# Autodesk Inventor assembly: Assembly_FINAL
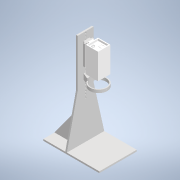
[picture p0: Inventor's stored thumbnail of the model, 180x180]
Saved by Autodesk Inventor 2021.2 (Build 252289000, 289)
## iProperties
Created: 2021-03-24
Part Number: Assembly_FINAL
Document SubType Name: Assembly
Designer: yxion
Author: yxion
## Documents named in this file (9)
- C:\Users\yxion\Documents\6_VandyUndergrad\4_ProgramManagement\EVD\CAD\Assembly_FINAL.iam
- C:\Users\yxion\Documents\6_VandyUndergrad\4_ProgramManagement\EVD\CAD\mdf_base_6x6.ipt
- C:\Users\yxion\Documents\6_VandyUndergrad\4_ProgramManagement\EVD\CAD\camera.ipt
- C:\Users\yxion\Documents\6_VandyUndergrad\4_ProgramManagement\EVD\CAD\mdf_support.ipt
- C:\Users\yxion\Documents\6_VandyUndergrad\4_ProgramManagement\EVD\CAD\5mm_bolt.ipt
- C:\Users\yxion\Documents\6_VandyUndergrad\4_ProgramManagement\EVD\CAD\ring_light_holder.ipt
- C:\Users\yxion\Documents\6_VandyUndergrad\4_ProgramManagement\EVD\CAD\mdf_vertical_r1.ipt
- C:\Users\yxion\Documents\6_VandyUndergrad\4_ProgramManagement\EVD\CAD\5mm_bolt_short.ipt
- C:\Users\yxion\Documents\6_VandyUndergrad\4_ProgramManagement\EVD\CAD\spacer_final.ipt
## Components (11 placed, 8 different names)
1. mdf_base_6x6:1 — Mate:10, Mate:13, Mate:15, Mate:16, Flush:2, Mate:17, Mate:18, Mate:19, Mate:20
2. camera:1 — Mate:30, Mate:42, Flush:3, Mate:43
3. mdf_support:1 — Mate:15, Mate:16, Mate:19
4. mdf_support:2 — Mate:10, Mate:13, Mate:20
5. 5mm_bolt:3 — Mate:26, Mate:28, Mate:30
6. 5mm_bolt:4 — Mate:25, Mate:27
7. ring_light_holder:1 — Mate:36, Mate:41
8. mdf_vertical_r1:1 — Flush:2, Mate:17, Mate:18, Mate:25, Mate:26, Mate:27, Mate:28, Mate:36, Mate:37, Mate:38, Mate:39, Mate:40
9. 5mm_bolt_short:1 — Mate:37, Mate:39, Mate:41
10. 5mm_bolt_short:2 — Mate:38, Mate:40
11. spacer_final:1 — Mate:42, Flush:3, Mate:43
## Relationships (23: Mate 21, Flush 2)
- Mate:10: mdf_base_6x6:1 ↔ mdf_support:2
- Mate:13: mdf_base_6x6:1 ↔ mdf_support:2
- Mate:15: mdf_base_6x6:1 ↔ mdf_support:1
- Mate:16: mdf_base_6x6:1 ↔ mdf_support:1
- Flush:2: mdf_base_6x6:1 ↔ mdf_vertical_r1:1
- Mate:17: mdf_base_6x6:1 ↔ mdf_vertical_r1:1
- Mate:18: mdf_base_6x6:1 ↔ mdf_vertical_r1:1
- Mate:19: mdf_base_6x6:1 ↔ mdf_support:1
- Mate:20: mdf_base_6x6:1 ↔ mdf_support:2
- Mate:25: 5mm_bolt:4 ↔ mdf_vertical_r1:1
- Mate:26: 5mm_bolt:3 ↔ mdf_vertical_r1:1
- Mate:27: 5mm_bolt:4 ↔ mdf_vertical_r1:1
- Mate:28: 5mm_bolt:3 ↔ mdf_vertical_r1:1
- Mate:30: camera:1 ↔ 5mm_bolt:3
- Mate:36: ring_light_holder:1 ↔ mdf_vertical_r1:1
- Mate:37: mdf_vertical_r1:1 ↔ 5mm_bolt_short:1
- Mate:38: mdf_vertical_r1:1 ↔ 5mm_bolt_short:2
- Mate:39: mdf_vertical_r1:1 ↔ 5mm_bolt_short:1
- Mate:40: mdf_vertical_r1:1 ↔ 5mm_bolt_short:2
- Mate:41: ring_light_holder:1 ↔ 5mm_bolt_short:1
- Mate:42: camera:1 ↔ spacer_final:1
- Flush:3: camera:1 ↔ spacer_final:1
- Mate:43: camera:1 ↔ spacer_final:1
